# Autodesk Inventor assembly: STEEL FRAME & RAILS ASSY
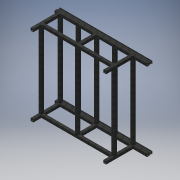
[picture p0: Inventor's stored thumbnail of the model, 180x180]
Saved by Autodesk Inventor 2018 (Build 220112000, 112)
## iProperties
Created: 2018-10-15
Part Number: STEEL FRAME & RAILS ASSY
Material: Genérico
Document SubType Name: Assembly
Designer: Toshiba
Author: Toshiba
## Documents named in this file (4)
- C:\U\Semestre Primavera 2018\Diseño de sistemas mecánicos\CNC\DiseñoCNC\Gantry\STEEL FRAME & RAILS ASSY.iam
- C:\U\Semestre Primavera 2018\Diseño de sistemas mecánicos\CNC\DiseñoCNC\Frame\STEEL FRAME ASSY.iam
- C:\U\Semestre Primavera 2018\Diseño de sistemas mecánicos\CNC\DiseñoCNC\Gantry\2570 STEEL PROFILE 60X40X2.ipt
- C:\U\Semestre Primavera 2018\Diseño de sistemas mecánicos\CNC\DiseñoCNC\Gantry\HDG RAIL.ipt
## Components (5 placed, 3 different names)
1. STEEL FRAME ASSY:1 [sub-assembly] — Coincidencia:1, Coincidencia:3, Coincidencia:4, Coincidencia:5, Coincidencia:6, Coincidencia:7, Coincidencia:8
2. 2570 STEEL PROFILE 60X40X2:1 — Coincidencia:1, Coincidencia:3, Coincidencia:8, Coincidencia:12, Coincidencia:13, Coincidencia:14, Insertar:2
3. 2570 STEEL PROFILE 60X40X2:2 — Coincidencia:4, Coincidencia:5, Coincidencia:6, Coincidencia:7, Coincidencia:9, Coincidencia:10, Coincidencia:11, Insertar:1
4. HDG RAIL:1 — Coincidencia:9, Coincidencia:10, Coincidencia:11, Insertar:1
5. HDG RAIL:2 — Coincidencia:12, Coincidencia:13, Coincidencia:14, Insertar:2
## Relationships (15: Mate 13, Insert 2)
- Coincidencia:1 [Mate]: STEEL FRAME ASSY:1 ↔ 2570 STEEL PROFILE 60X40X2:1
- Coincidencia:3 [Mate]: STEEL FRAME ASSY:1 ↔ 2570 STEEL PROFILE 60X40X2:1
- Coincidencia:4 [Mate]: STEEL FRAME ASSY:1 ↔ 2570 STEEL PROFILE 60X40X2:2
- Coincidencia:5 [Mate]: STEEL FRAME ASSY:1 ↔ 2570 STEEL PROFILE 60X40X2:2
- Coincidencia:6 [Mate]: STEEL FRAME ASSY:1 ↔ 2570 STEEL PROFILE 60X40X2:2
- Coincidencia:7 [Mate] (17.5 mm): STEEL FRAME ASSY:1 ↔ 2570 STEEL PROFILE 60X40X2:2
- Coincidencia:8 [Mate] (17.5 mm): STEEL FRAME ASSY:1 ↔ 2570 STEEL PROFILE 60X40X2:1
- Coincidencia:9 [Mate]: 2570 STEEL PROFILE 60X40X2:2 ↔ HDG RAIL:1
- Coincidencia:10 [Mate]: 2570 STEEL PROFILE 60X40X2:2 ↔ HDG RAIL:1
- Coincidencia:11 [Mate]: 2570 STEEL PROFILE 60X40X2:2 ↔ HDG RAIL:1
- Insertar:1: 2570 STEEL PROFILE 60X40X2:2 ↔ HDG RAIL:1
- Coincidencia:12 [Mate]: 2570 STEEL PROFILE 60X40X2:1 ↔ HDG RAIL:2
- Coincidencia:13 [Mate]: 2570 STEEL PROFILE 60X40X2:1 ↔ HDG RAIL:2
- Coincidencia:14 [Mate]: 2570 STEEL PROFILE 60X40X2:1 ↔ HDG RAIL:2
- Insertar:2: 2570 STEEL PROFILE 60X40X2:1 ↔ HDG RAIL:2
